# Autodesk Inventor assembly: LegUpperFrontLinkUnit
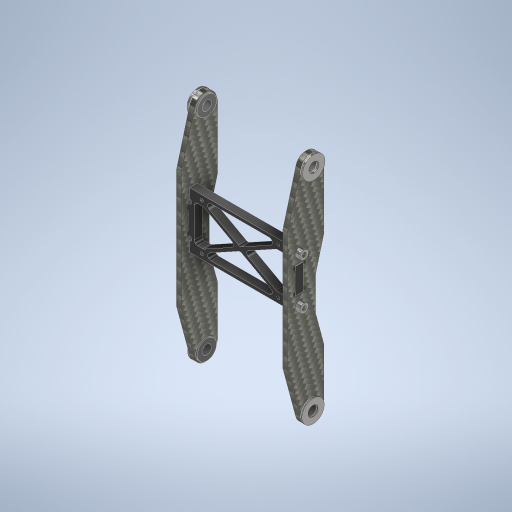
[picture p0: Inventor's stored thumbnail of the model, 512x512]
Saved by Autodesk Inventor 2024.2 (Build 282272000, 272)
## iProperties
Created: 2024-01-05
Part Number: LegUpperFrontLinkUnit
Document SubType Name: Assembly
Designer: Masato Kubotera
Mass: 41.2321 g
Surface Area: 218.625 cm^2
Volume: 20.906 cm^3
Density: 1.97226 g/cm^3
Author: Masato Kubotera
## Documents named in this file (8)
- D:\OneDrive - Chiba Institute of Technology\CIT Brains\RoboCup2024\Mechanic\SUSTAINA-OP2-DEV\NativeFiles\Boby\LowerLimb\Legs\Links\LegUpperFrontLinkUnit.iam
- D:\OneDrive - Chiba Institute of Technology\CIT Brains\RoboCup2024\Mechanic\SUSTAINA-OP2-DEV\NativeFiles\Boby\LowerLimb\Legs\Links\LegLinkBraceFrame.ipt
- D:\OneDrive - Chiba Institute of Technology\CIT Brains\RoboCup2024\Mechanic\SUSTAINA-OP2-DEV\NativeFiles\Boby\LowerLimb\Legs\Links\LegFrontLinkFrame.ipt
- D:\OneDrive - Chiba Institute of Technology\CIT Brains\RoboCup2024\Mechanic\SUSTAINA-OP2-DEV\NativeFiles\Boby\COTS\Bushes\GFM-0608-04.ipt
- D:\OneDrive - Chiba Institute of Technology\CIT Brains\RoboCup2024\Mechanic\SUSTAINA-OP2-DEV\NativeFiles\Boby\COTS\Screws\CapScrew\UC-0308.ipt
- D:\OneDrive - Chiba Institute of Technology\CIT Brains\RoboCup2024\Mechanic\SUSTAINA-OP2-DEV\NativeFiles\Boby\COTS\Washers\Metal\UUW-0614-05H.ipt
- D:\OneDrive - Chiba Institute of Technology\CIT Brains\RoboCup2024\Mechanic\SUSTAINA-OP2-DEV\NativeFiles\Boby\COTS\Washers\Metal\UUW-0614-10H.ipt
- D:\OneDrive - Chiba Institute of Technology\CIT Brains\RoboCup2024\Mechanic\SUSTAINA-OP2-DEV\NativeFiles\Boby\COTS\Washers\Resin\TT-0614-05.ipt
## Components (19 placed, 7 different names)
1. LegLinkBraceFrame:1 — Insert:1, Insert:2, Flush:1, Angle:1, Insert:13, Insert:14
2. LegFrontLinkFrame:1 — Insert:13, Insert:14, Insert:15, Insert:16, Insert:19, Insert:20, Insert:21, Insert:22
3. LegFrontLinkFrame:2 — Insert:1, Insert:2, Insert:5, Insert:6, Insert:7, Insert:8, Insert:11, Insert:12
4. GFM-0608-04:1 — Insert:5
5. GFM-0608-04:2 — Insert:6, Mate:1
6. GFM-0608-04:3 — Insert:15
7. GFM-0608-04:4 — Insert:16
8. UC-0308:1 — Insert:11
9. UC-0308:2 — Insert:12
10. UC-0308:3 — Insert:21
11. UC-0308:4 — Insert:22
12. TT-0614-05:1 — Insert:7, Insert:9
13. TT-0614-05:1 — Insert:8, Insert:10
14. TT-0614-05:2 — Insert:19
15. TT-0614-05:2 — Insert:20
16. UUW-0614-10H:1 — Insert:9
17. UUW-0614-05H:2 — Insert:10
18. UUW-0614-10H:2
19. UUW-0614-05H:4
## Relationships (23: Insert 20, Mate 1, Flush 1, Angle 1)
- Insert:1: LegLinkBraceFrame:1 ↔ LegFrontLinkFrame:2
- Insert:2: LegLinkBraceFrame:1 ↔ LegFrontLinkFrame:2
- Mate:1: GFM-0608-04:2
- Flush:1: LegLinkBraceFrame:1
- Angle:1 (0 deg): LegLinkBraceFrame:1
- Insert:5: LegFrontLinkFrame:2 ↔ GFM-0608-04:1
- Insert:6: LegFrontLinkFrame:2 ↔ GFM-0608-04:2
- Insert:7: LegFrontLinkFrame:2 ↔ TT-0614-05:1
- Insert:8: LegFrontLinkFrame:2 ↔ TT-0614-05:1
- Insert:9: TT-0614-05:1 ↔ UUW-0614-10H:1
- Insert:10: TT-0614-05:1 ↔ UUW-0614-05H:2
- Insert:11: LegFrontLinkFrame:2 ↔ UC-0308:1
- Insert:12: LegFrontLinkFrame:2 ↔ UC-0308:2
- Insert:13: LegLinkBraceFrame:1 ↔ LegFrontLinkFrame:1
- Insert:14: LegLinkBraceFrame:1 ↔ LegFrontLinkFrame:1
- Insert:15: LegFrontLinkFrame:1 ↔ GFM-0608-04:3
- Insert:16: LegFrontLinkFrame:1 ↔ GFM-0608-04:4
- [Insert]: TT-0614-05:2 ↔ UUW-0614-10H:2
- [Insert]: TT-0614-05:2 ↔ UUW-0614-05H:4
- Insert:19: LegFrontLinkFrame:1 ↔ TT-0614-05:2
- Insert:20: LegFrontLinkFrame:1 ↔ TT-0614-05:2
- Insert:21: LegFrontLinkFrame:1 ↔ UC-0308:3
- Insert:22: LegFrontLinkFrame:1 ↔ UC-0308:4
## Named parameters: d19_d11 = 0 mm, d20_d11 = 0 mm
